# Autodesk Inventor assembly: MagnetAssembly
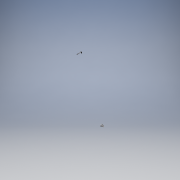
[picture p0: Inventor's stored thumbnail of the model, 180x180]
Saved by Autodesk Inventor 2017 (Build 210142000, 142)
## iProperties
Created: 2016-12-31
Part Number: MagnetAssembly
Document SubType Name: Assembly
Designer: umr
Author: umr
## Documents named in this file (8)
- D:\SeniorProject\Models2\UTM\MagnetAssembly.iam
- D:\SeniorProject\Models2\UTM\M3 Screw_30mm.ipt
- D:\SeniorProject\Models2\UTM\M3 Spring 94125K472.ipt
- D:\SeniorProject\Models2\UTM\M3 Locknut.ipt
- D:\SeniorProject\Models2\UTM\Zip Tie.ipt
- D:\SeniorProject\Models2\UTM\15mm x 5mm x 5mm Ring Magnet.ipt
- D:\SeniorProject\Models2\UTM\M5 Screw_16mm.ipt
- D:\SeniorProject\Models2\UTM\M5 Locknut.ipt
## Components (7 placed, 7 different names)
1. M3 Spring 94125K472:1 — Mate:15, Mate:17
2. M3 Locknut:1 — Mate:18, Mate:21
3. M3 Screw_30mm:1 — Mate:15, Mate:17, Mate:18, Mate:20
4. Zip Tie:1 — Mate:20, Mate:21
5. 15mm x 5mm x 5mm Ring Magnet:1 — Mate:22, Mate:23
6. M5 Screw_16mm:1 — Mate:22, Mate:23, Mate:24, Flush:2
7. M5 Locknut:1 — Mate:24, Flush:2
## Relationships (9: Mate 8, Flush 1)
- Mate:15: M3 Spring 94125K472:1 ↔ M3 Screw_30mm:1
- Mate:17: M3 Spring 94125K472:1 ↔ M3 Screw_30mm:1
- Mate:18: M3 Locknut:1 ↔ M3 Screw_30mm:1
- Mate:20: M3 Screw_30mm:1 ↔ Zip Tie:1
- Mate:21: M3 Locknut:1 ↔ Zip Tie:1
- Mate:22: 15mm x 5mm x 5mm Ring Magnet:1 ↔ M5 Screw_16mm:1
- Mate:23: 15mm x 5mm x 5mm Ring Magnet:1 ↔ M5 Screw_16mm:1
- Mate:24: M5 Screw_16mm:1 ↔ M5 Locknut:1
- Flush:2 (2 mm): M5 Screw_16mm:1 ↔ M5 Locknut:1
